# Autodesk Inventor assembly: AssemblyForSketch
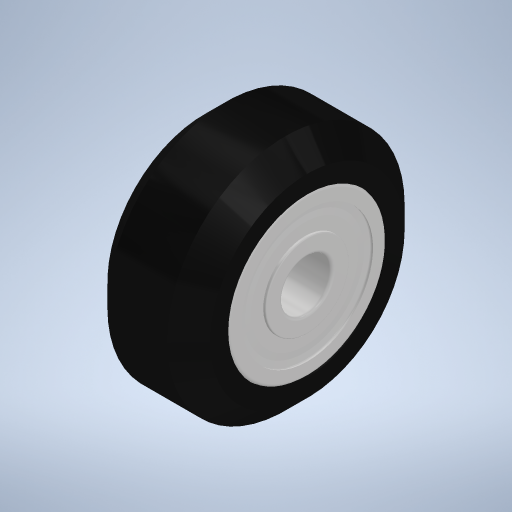
[picture p0: Inventor's stored thumbnail of the model, 512x512]
Saved by Autodesk Inventor 2024.2 (Build 282272000, 272)
## iProperties
Created: 2025-08-04
Part Number: AssemblyForSketch
Document SubType Name: Assembly
Designer: Admin
Author: 3:1
Title: Rodamiento Delrin V
Subject: 30???
## Documents named in this file (3)
- C:\Users\Admin\Documents\GitHub\ManipuladorCartesiano\DiseñoMecánico\AuxiliarPieces\Bearings\625ZZ\BearingAssemblyForSketch.iam
- C:\Users\Admin\Documents\GitHub\ManipuladorCartesiano\DiseñoMecánico\AuxiliarPieces\Bearings\625ZZ\Roldana V Nylon.ipt
- C:\Users\Admin\Documents\GitHub\ManipuladorCartesiano\DiseñoMecánico\AuxiliarPieces\Bearings\625ZZ\SKF_625_2Z v1.ipt
## Components (2 placed, 2 different names)
1. Roldana V Nylon:1 — Mate:1, Mate:2
2. SKF_625_2Z v1:1 — Mate:1, Mate:2
## Relationships (2: Mate 2)
- Mate:1: Roldana V Nylon:1 ↔ SKF_625_2Z v1:1
- Mate:2: Roldana V Nylon:1 ↔ SKF_625_2Z v1:1
